# Autodesk Inventor assembly: Drivetrain (Right)
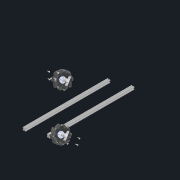
[picture p0: Inventor's stored thumbnail of the model, 180x180]
Saved by Autodesk Inventor 2022 (Build 260153000, 153)
## iProperties
Created: 2022-01-18
Part Number: Drivetrain (Right)
Document SubType Name: Assembly
Designer: divid
Author: divid
## Documents named in this file (5)
- C:\Users\divid\Documents\GitHub\ComputerAidedDesign\2021-22\FTC\#13822 Robovikes\Drivetrain\Drivetrain (Right).iam
- C:\Users\divid\Documents\GitHub\ComputerAidedDesign\2021-22\FTC\#13822 Robovikes\Drivetrain\15mm Extrusion - 420mm - 90° Ends.ipt
- C:\Users\divid\Documents\GitHub\ComputerAidedDesign\2021-22\FTC\#13822 Robovikes\Drivetrain\Wheel Assembly\Wheel Assembly (Left).iam
- C:\Users\divid\Documents\GitHub\ComputerAidedDesign\2021-22\FTC\#13822 Robovikes\Drivetrain\Wheel Assembly\Wheel Assembly (Right).iam
- C:\Users\divid\Documents\GitHub\ComputerAidedDesign\2021-22\FTC\#13822 Robovikes\Drivetrain\M3 x 8mm Hex Cap Screws.ipt
## Components (12 placed, 4 different names)
1. 15mm Extrusion - 420mm - 90° Ends:1
2. 15mm Extrusion - 420mm - 90° Ends:2
3. Wheel Assembly (Left):1 [sub-assembly] — Mate:1, Mate:2, Mate:3, Mate:4
4. Wheel Assembly (Right):1 [sub-assembly] — Mate:5, Mate:6, Mate:7, Mate:8
5. M3 x 8mm Hex Cap Screws:1 — Mate:2
6. M3 x 8mm Hex Cap Screws:2 — Mate:3
7. M3 x 8mm Hex Cap Screws:3 — Mate:4
8. M3 x 8mm Hex Cap Screws:4 — Mate:1
9. M3 x 8mm Hex Cap Screws:5 — Mate:6
10. M3 x 8mm Hex Cap Screws:6 — Mate:8
11. M3 x 8mm Hex Cap Screws:7 — Mate:5
12. M3 x 8mm Hex Cap Screws:8 — Mate:7
## Relationships (8: Mate 8)
- Mate:1: Wheel Assembly (Left):1 ↔ M3 x 8mm Hex Cap Screws:4
- Mate:2: Wheel Assembly (Left):1 ↔ M3 x 8mm Hex Cap Screws:1
- Mate:3: Wheel Assembly (Left):1 ↔ M3 x 8mm Hex Cap Screws:2
- Mate:4: Wheel Assembly (Left):1 ↔ M3 x 8mm Hex Cap Screws:3
- Mate:5: Wheel Assembly (Right):1 ↔ M3 x 8mm Hex Cap Screws:7
- Mate:6: Wheel Assembly (Right):1 ↔ M3 x 8mm Hex Cap Screws:5
- Mate:7: Wheel Assembly (Right):1 ↔ M3 x 8mm Hex Cap Screws:8
- Mate:8: Wheel Assembly (Right):1 ↔ M3 x 8mm Hex Cap Screws:6
